# Autodesk Inventor assembly: Assembly1
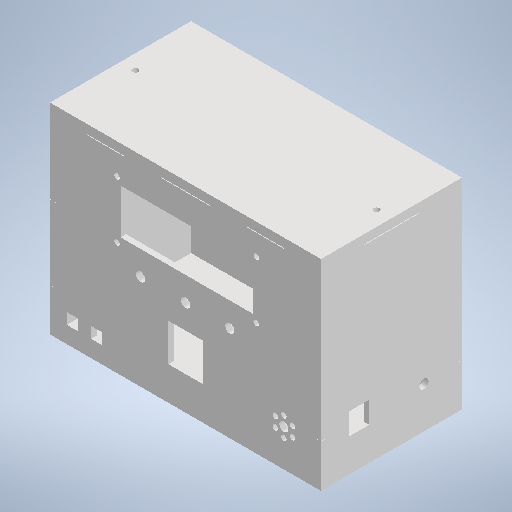
[picture p0: Inventor's stored thumbnail of the model, 512x512]
Saved by Autodesk Inventor 2025.2 (Build 292293000, 293)
## iProperties
Created: 2024-12-18
Part Number: Assembly1
Document SubType Name: Assembly
Designer: Inteli
Author: Inteli
## Documents named in this file (8)
- C:\Users\Inteli\OneDrive\Documentos\Assembly1.iam
- C:\Users\Inteli\OneDrive\Documentos\frente-case.ipt
- C:\Users\Inteli\OneDrive\Documentos\verso-case.ipt
- C:\Users\Inteli\OneDrive\Documentos\cima-case-1.ipt
- C:\Users\Inteli\OneDrive\Documentos\cima-case-2.ipt
- C:\Users\Inteli\OneDrive\Documentos\base-case.ipt
- C:\Users\Inteli\OneDrive\Documentos\lado-direito-case.ipt
- C:\Users\Inteli\OneDrive\Documentos\lado-esquerdo-case.ipt
## Components (7 placed, 7 different names)
1. frente-case:1 — Flush:7, Flush:8, Flush:9, Flush:15
2. verso-case:1 — Flush:10, Flush:11, Flush:12
3. cima-case-1:1 — Flush:13, Flush:14, Flush:15, Mate:1, Mate:2
4. cima-case-2:1 — Mate:1, Mate:2
5. base-case:1 — Flush:1, Flush:2, Flush:3, Flush:4, Flush:5, Flush:6, Flush:7, Flush:8, Flush:10, Flush:12
6. lado-direito-case:1 — Flush:1, Flush:2, Flush:3, Flush:13
7. lado-esquerdo-case:1 — Flush:4, Flush:5, Flush:6, Flush:9, Flush:11, Flush:14
## Relationships (17: Flush 15, Mate 2)
- Flush:1: base-case:1 ↔ lado-direito-case:1
- Flush:2: base-case:1 ↔ lado-direito-case:1
- Flush:3: base-case:1 ↔ lado-direito-case:1
- Flush:4: base-case:1 ↔ lado-esquerdo-case:1
- Flush:5: base-case:1 ↔ lado-esquerdo-case:1
- Flush:6: base-case:1 ↔ lado-esquerdo-case:1
- Flush:7: frente-case:1 ↔ base-case:1
- Flush:8: frente-case:1 ↔ base-case:1
- Flush:9: frente-case:1 ↔ lado-esquerdo-case:1
- Flush:10: verso-case:1 ↔ base-case:1
- Flush:11: verso-case:1 ↔ lado-esquerdo-case:1
- Flush:12: verso-case:1 ↔ base-case:1
- Flush:13: cima-case-1:1 ↔ lado-direito-case:1
- Flush:14: cima-case-1:1 ↔ lado-esquerdo-case:1
- Flush:15: frente-case:1 ↔ cima-case-1:1
- Mate:1: cima-case-1:1 ↔ cima-case-2:1
- Mate:2: cima-case-1:1 ↔ cima-case-2:1
